# Autodesk Inventor assembly: Компоновка
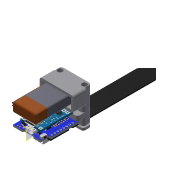
[picture p0: Inventor's stored thumbnail of the model, 180x180]
Saved by Autodesk Inventor 2021 (Build 250183000, 183)
## iProperties
Created: 2023-02-18
Part Number: Компоновка
Document SubType Name: Assembly
Designer: Tasya
Mass: 23.563 g
Surface Area: 176.471 cm^2
Volume: 17.7887 cm^3
Density: 1.3246 g/cm^3
Author: Tasya
## Documents named in this file (9)
- C:\Users\Tasya\Desktop\теплица\3D\Сборки iam\Компоновка.iam
- C:\Users\Tasya\Desktop\теплица\grabcad\Wemos_D1_mini.ipt
- C:\Users\Tasya\Desktop\теплица\датчики почва воздух\Кронштейн МК.ipt
- C:\Users\Tasya\Desktop\теплица\grabcad\Capacative Soil Moisture Sensor.ipt
- C:\Users\Tasya\Desktop\теплица\датчики почва воздух\Пластина.ipt
- C:\Users\Tasya\Documents\Inventor\Content Center Files\R2021\ru-RU\Screw GOST R 2009-2013\Screw A.M2-6gx8 GOST R 50403-92(1).ipt
- C:\Users\Tasya\Desktop\теплица\grabcad\TP4056_Charging_Module_Type_C.iam
- C:\Users\Tasya\Desktop\теплица\датчики почва воздух\Кронштейн АКБ.ipt
- C:\Users\Tasya\Desktop\теплица\grabcad\Li-po.ipt
## Components (9 placed, 8 different names)
1. Wemos_D1_mini:1 — Совмещение:1, Совмещение:2, Совмещение:3, Заподлицо:1, Заподлицо:11
2. Кронштейн МК:1 — Заподлицо:1, Совмещение:6, Заподлицо:12
3. Capacative Soil Moisture Sensor:1 — Угол:1, Заподлицо:5, Заподлицо:6, Заподлицо:7
4. Пластина:1 — Заподлицо:6, Заподлицо:7, Совмещение:4, Совмещение:5, Заподлицо:9
5. Screw GOST R 2009-2013 M2x8-A:1 — Совмещение:4, Заподлицо:8
6. Screw GOST R 2009-2013 M2x8-A:2 — Совмещение:5, Заподлицо:8, Заподлицо:9
7. TP4056_Charging_Module_Type_C:1 [sub-assembly] — Совмещение:6, Заподлицо:10, Заподлицо:11
8. Кронштейн АКБ:1 — Заподлицо:12, Совмещение:7, Совмещение:9
9. Li-po:1 — Совмещение:7, Совмещение:8, Совмещение:9
## Relationships (19: Mate 9, Flush 9, Angle 1)
- Совмещение:1 [Mate]: Wemos_D1_mini:1
- Совмещение:2 [Mate]: Wemos_D1_mini:1
- Совмещение:3 [Mate]: Wemos_D1_mini:1
- Заподлицо:1 [Flush]: Wemos_D1_mini:1 ↔ Кронштейн МК:1
- Угол:1 [Angle] (180 deg): Capacative Soil Moisture Sensor:1
- Заподлицо:5 [Flush]: Capacative Soil Moisture Sensor:1
- Заподлицо:6 [Flush]: Capacative Soil Moisture Sensor:1 ↔ Пластина:1
- Заподлицо:7 [Flush]: Capacative Soil Moisture Sensor:1 ↔ Пластина:1
- Совмещение:4 [Mate]: Пластина:1 ↔ Screw GOST R 2009-2013 M2x8-A:1
- Совмещение:5 [Mate]: Пластина:1 ↔ Screw GOST R 2009-2013 M2x8-A:2
- Заподлицо:8 [Flush]: Screw GOST R 2009-2013 M2x8-A:1 ↔ Screw GOST R 2009-2013 M2x8-A:2
- Заподлицо:9 [Flush]: Пластина:1 ↔ Screw GOST R 2009-2013 M2x8-A:2
- Совмещение:6 [Mate]: Кронштейн МК:1 ↔ TP4056_Charging_Module_Type_C:1
- Заподлицо:10 [Flush]: TP4056_Charging_Module_Type_C:1
- Заподлицо:11 [Flush]: Wemos_D1_mini:1 ↔ TP4056_Charging_Module_Type_C:1
- Заподлицо:12 [Flush]: Кронштейн МК:1 ↔ Кронштейн АКБ:1
- Совмещение:7 [Mate]: Кронштейн АКБ:1 ↔ Li-po:1
- Совмещение:8 [Mate]: Li-po:1
- Совмещение:9 [Mate]: Кронштейн АКБ:1 ↔ Li-po:1
